# Autodesk Inventor assembly: 2024_0222_KickerParts
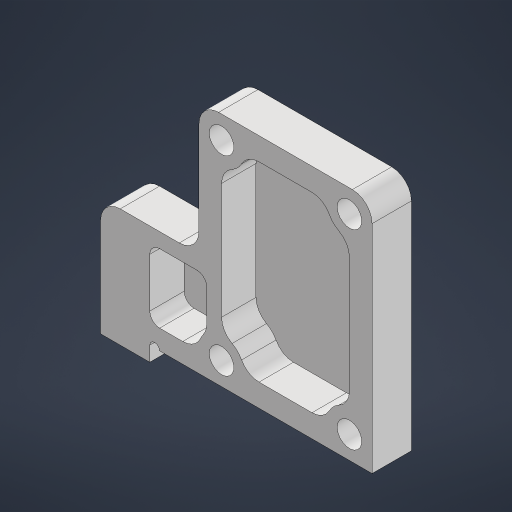
[picture p0: Inventor's stored thumbnail of the model, 512x512]
Saved by Autodesk Inventor 2024.2 (Build 282272000, 272)
## iProperties
Created: 2024-02-22
Part Number: 2024_0222_KickerParts
Document SubType Name: Assembly
Designer: Hanaoka
Author: Hanaoka
## Documents named in this file (2)
- G:\共有ドライブ\reRo\05_個人\hanaoka\inventor\CAMpath\2024_0222_KickerParts.iam
- G:\共有ドライブ\reRo\05_個人\hanaoka\inventor\KickerUnit\SolenoidMount.ipt
## Components (1 placed, 1 different names)
1. SolenoidMount:1 — メイト:1, メイト:2, メイト:3
## Relationships (3: Mate 3)
- メイト:1 [Mate]: SolenoidMount:1
- メイト:2 [Mate]: SolenoidMount:1
- メイト:3 [Mate]: SolenoidMount:1
